# Autodesk Inventor assembly: Ammonia Filter Tub
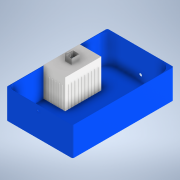
[picture p0: Inventor's stored thumbnail of the model, 180x180]
Saved by Autodesk Inventor 2020 (Build 240168000, 168)
## iProperties
Created: 2020-08-17
Part Number: Ammonia Filter Tub
Document SubType Name: Assembly
Designer: Abbas
Author: Abbas
## Documents named in this file (5)
- C:\Users\LENOVO\Desktop\Graduation Project\Fish Farming Unit\Ammonia Filter Tub\Ammonia Filter Tub.iam
- C:\Users\LENOVO\Desktop\Graduation Project\Fish Farming Unit\Ammonia Filter Tub\Ammonia Filter Tub.ipt
- C:\Users\LENOVO\Desktop\Graduation Project\Fish Farming Unit\Ammonia Filter Sensor Holder\Ammonia Filter Sensor Holder.ipt
- C:\Users\LENOVO\Desktop\Graduation Project\Fish Farming Unit\Feeding Mechanism\HC-SR04_ultrasonic.iam
- C:\Users\LENOVO\Desktop\Graduation Project\Fish Farming Unit\Gland\pg7.ipt
## Components (4 placed, 4 different names)
1. Ammonia Filter Tub:2 — Mate:1, Mate:2
2. Ammonia Filter Sensor Holder:1 — Mate:1, Mate:2, Insert:1, Insert:2
3. HC-SR04_ultrasonic:2 [sub-assembly] — Insert:1
4. pg7:1 — Insert:2
## Relationships (4: Mate 2, Insert 2)
- Mate:1: Ammonia Filter Tub:2 ↔ Ammonia Filter Sensor Holder:1
- Mate:2: Ammonia Filter Tub:2 ↔ Ammonia Filter Sensor Holder:1
- Insert:1 (-5 mm): Ammonia Filter Sensor Holder:1 ↔ HC-SR04_ultrasonic:2
- Insert:2 (-9.5 mm): Ammonia Filter Sensor Holder:1 ↔ pg7:1
